# Autodesk Inventor assembly: Ring Mod
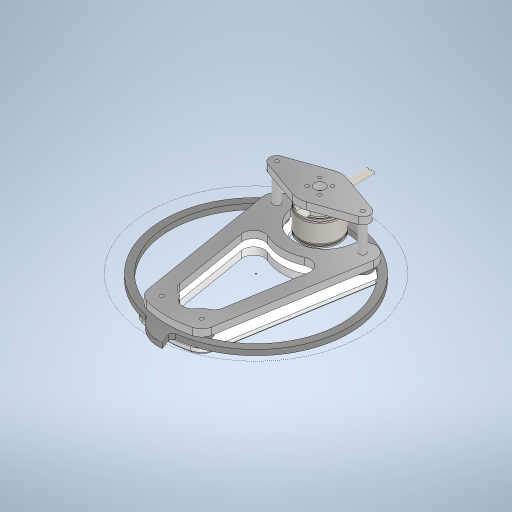
[picture p0: Inventor's stored thumbnail of the model, 512x512]
Saved by Autodesk Inventor 2023.2 (Build 272271000, 271)
## iProperties
Created: 2023-10-14
Part Number: Ring Mod
Document SubType Name: Assembly
Designer: Nathan Cai
Mass: 399.8 g
Surface Area: 572.576 cm^2
Volume: 91.5051 cm^3
Density: 4.36915 g/cm^3
Author: Nathan Cai
## Documents named in this file (9)
- E:\Documents\Inventor\Law - V2.0\Hori - Ring\Ring Mod.iam
- E:\Documents\Inventor\Law - V2.0\Hori - Ring\Upright - Lower.ipt
- E:\Documents\Inventor\Law - V2.0\Hori - Ring\Standoff 1in.ipt
- E:\Documents\Inventor\Law - V2.0\Hori - Ring\Standoff 0.25in.ipt
- E:\Documents\Inventor\Law - V2.0\Hori - Ring\5-8in OD Ball Bearing.ipt
- E:\Documents\Inventor\Law - V2.0\Hori - Ring\Blade - Ring.ipt
- E:\Documents\Inventor\Law - V2.0\Hori - Ring\Part5.ipt
- E:\Documents\Inventor\Law - V2.0\Hori - Ring\Upright - Top.ipt
- E:\Documents\Inventor\Law - V2.0\Hori - Ring\Upright - Brace.ipt
## Components (15 placed, 8 different names)
1. Upright - Lower:1 — Mate:1, Mate:2, Mate:3, Mate:4, Mate:5, Mate:6, Mate:7, Mate:8, Mate:13, Mate:14, Mate:15, Mate:16, Mate:17, Mate:23, Mate:24
2. Standoff 1in:1 — Mate:1, Mate:3, Mate:21
3. Standoff 1in:2 — Mate:2, Mate:4, Flush:5, Mate:20
4. Standoff 0.25in:1 — Mate:5, Mate:7, Mate:9, Flush:3
5. Standoff 0.25in:2 — Mate:6, Mate:8, Mate:10
6. 5-8in OD Ball Bearing:1 — Mate:9, Flush:2, Flush:3, Flush:4, Tangent:1
7. 5-8in OD Ball Bearing:2 — Mate:10, Flush:2, Tangent:2
8. Standoff 0.25in:3 — Mate:13, Mate:15
9. 5-8in OD Ball Bearing:3 — Flush:1, Flush:4, Tangent:3
10. Standoff 0.25in:4 — Mate:14, Mate:16, Mate:25
11. 5-8in OD Ball Bearing:4 — Flush:1, Tangent:4
12. Blade - Ring:1 — Tangent:1, Tangent:2, Mate:17, Tangent:3, Tangent:4
13. Part5:1 — Flush:5, Mate:18, Mate:19, Mate:22
14. Upright - Top:1 — Mate:18, Mate:19, Mate:20, Mate:21, Mate:22
15. Upright - Brace:1 — Mate:23, Mate:24, Mate:25
## Relationships (34: Mate 25, Flush 5, Tangent 4)
- Mate:1: Upright - Lower:1 ↔ Standoff 1in:1
- Mate:2: Upright - Lower:1 ↔ Standoff 1in:2
- Mate:3: Upright - Lower:1 ↔ Standoff 1in:1
- Mate:4: Upright - Lower:1 ↔ Standoff 1in:2
- Mate:5: Upright - Lower:1 ↔ Standoff 0.25in:1
- Mate:6: Upright - Lower:1 ↔ Standoff 0.25in:2
- Mate:7: Upright - Lower:1 ↔ Standoff 0.25in:1
- Mate:8: Upright - Lower:1 ↔ Standoff 0.25in:2
- Mate:9: Standoff 0.25in:1 ↔ 5-8in OD Ball Bearing:1
- Mate:10: Standoff 0.25in:2 ↔ 5-8in OD Ball Bearing:2
- [Mate]: Standoff 0.25in:3 ↔ 5-8in OD Ball Bearing:3
- [Mate]: Standoff 0.25in:4 ↔ 5-8in OD Ball Bearing:4
- Mate:13: Upright - Lower:1 ↔ Standoff 0.25in:3
- Mate:14: Upright - Lower:1 ↔ Standoff 0.25in:4
- Mate:15: Upright - Lower:1 ↔ Standoff 0.25in:3
- Mate:16: Upright - Lower:1 ↔ Standoff 0.25in:4
- Flush:1: 5-8in OD Ball Bearing:3 ↔ 5-8in OD Ball Bearing:4
- Flush:2: 5-8in OD Ball Bearing:1 ↔ 5-8in OD Ball Bearing:2
- Flush:3 (-0.6858 mm): Standoff 0.25in:1 ↔ 5-8in OD Ball Bearing:1
- Flush:4: 5-8in OD Ball Bearing:1 ↔ 5-8in OD Ball Bearing:3
- Tangent:1: 5-8in OD Ball Bearing:1 ↔ Blade - Ring:1
- Tangent:2: 5-8in OD Ball Bearing:2 ↔ Blade - Ring:1
- Mate:17 (0.7937 mm): Upright - Lower:1 ↔ Blade - Ring:1
- Tangent:3: 5-8in OD Ball Bearing:3 ↔ Blade - Ring:1
- Tangent:4: 5-8in OD Ball Bearing:4 ↔ Blade - Ring:1
- Flush:5: Standoff 1in:2 ↔ Part5:1
- Mate:18: Part5:1 ↔ Upright - Top:1
- Mate:19: Part5:1 ↔ Upright - Top:1
- Mate:20: Standoff 1in:2 ↔ Upright - Top:1
- Mate:21: Standoff 1in:1 ↔ Upright - Top:1
- Mate:22: Part5:1 ↔ Upright - Top:1
- Mate:23: Upright - Lower:1 ↔ Upright - Brace:1
- Mate:24: Upright - Lower:1 ↔ Upright - Brace:1
- Mate:25: Standoff 0.25in:4 ↔ Upright - Brace:1
## Named parameters: d10_d8 = 0 mm, d11_d8 = 0 mm
